# Autodesk Inventor assembly: Assembly6
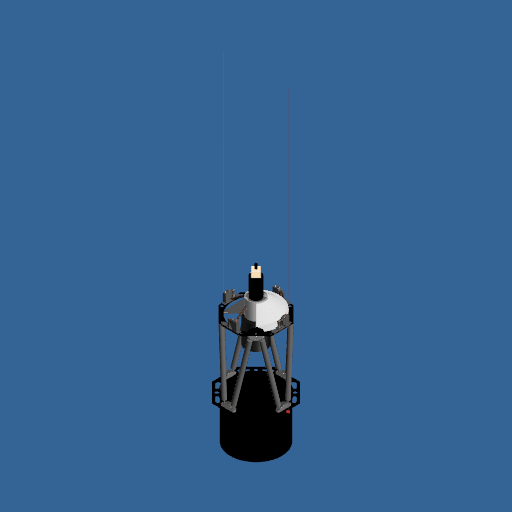
[picture p0: Inventor's stored thumbnail of the model, 512x512]
Saved by Autodesk Inventor 2026.2 (Build 302298000, 298)
## iProperties
Created: 2025-12-09
Part Number: Assembly6
Document SubType Name: Assembly
Designer: Thoma
Mass: 27295.5 g
Surface Area: 25498 cm^2
Volume: 10830.6 cm^3
Density: 2.52023 g/cm^3
Author: Thoma
## Documents named in this file (30)
- C:\Users\Thoma\OneDrive\Desktop\dir\telescope_cover\cover\derive_covers_v4.iam
- C:\Users\Thoma\OneDrive\Desktop\dir\telescope_cover\telescope\version_3\Telescope_End.ipt
- C:\Users\Thoma\OneDrive\Desktop\dir\telescope_cover\telescope\version_3\Triangle.ipt
- C:\Users\Thoma\OneDrive\Desktop\dir\telescope_cover\telescope\version_3\Triangle_Bracket_Top.ipt
- C:\Users\Thoma\OneDrive\Desktop\dir\telescope_cover\telescope\version_3\Carbon_Fibre.ipt
- C:\Users\Thoma\OneDrive\Desktop\dir\telescope_cover\telescope\version_3\5mm Screw.ipt
- C:\Users\Thoma\OneDrive\Desktop\dir\telescope_cover\telescope\version_3\35mm_bolt.ipt
- C:\Users\Thoma\OneDrive\Desktop\dir\telescope_cover\telescope\version_3\Triangle_Bracket_Bottom_MIR.ipt
- C:\Users\Thoma\OneDrive\Desktop\dir\telescope_cover\telescope\version_3\Telescope_Base.ipt
- C:\Users\Thoma\OneDrive\Desktop\dir\telescope_cover\telescope\version_3\Full_shaft_Simplify_3.ipt
- C:\Users\Thoma\OneDrive\Desktop\dir\telescope_cover\cover\Conic_Cover_Simplify_1.ipt
- C:\Users\Thoma\OneDrive\Desktop\dir\telescope_cover\telescope\version_3\30mm_bolt.ipt
- C:\Users\Thoma\OneDrive\Desktop\dir\telescope_cover\telescope\version_3\Baffle.ipt
- C:\Users\Thoma\OneDrive\Desktop\dir\telescope_cover\telescope\version_3\Bottom_End_Top.ipt
- C:\Users\Thoma\OneDrive\Desktop\dir\telescope_cover\cover\Cover_Upper_v3.ipt
- C:\Users\Thoma\OneDrive\Desktop\dir\telescope_cover\telescope\version_3\Laser.ipt
- C:\Users\Thoma\OneDrive\Desktop\dir\telescope_cover\cover\rod_v10.ipt
- C:\Users\Thoma\OneDrive\Desktop\dir\telescope_cover\servo\DSS-M15S Servo.ipt
- C:\Users\Thoma\OneDrive\Desktop\dir\telescope_cover\cover\Base_Plate_bottom.ipt
- C:\Users\Thoma\OneDrive\Desktop\dir\telescope_cover\cover\pawn.ipt
- C:\Users\Thoma\OneDrive\Desktop\dir\telescope_cover\cover\4mm_screw.ipt
- C:\Users\Thoma\OneDrive\Desktop\dir\telescope_cover\cover\6mm_washer_1mm.ipt
- C:\Users\Thoma\OneDrive\Desktop\dir\telescope_cover\cover\base_plate_v8.ipt
- C:\Users\Thoma\OneDrive\Desktop\dir\telescope_cover\screws\M2_Insert.ipt
- C:\Users\Thoma\OneDrive\Desktop\dir\telescope_cover\screws\Screw_DIN_912_M2x5F_A2.ipt
- C:\Users\Thoma\OneDrive\Desktop\dir\telescope_cover\screws\washer_bossard_m2-5_1170171.ipt
- C:\Users\Thoma\OneDrive\Desktop\dir\telescope_cover\screws\m4 threaded insert\m4 threaded insert\m4 threaded insert.ipt
- C:\Users\Thoma\OneDrive\Desktop\dir\telescope_cover\screws\M4 Washer - 9.0 x 0.9 - Black\M4 Washer - 9.0 x 0.9 - Black\M4 Washer - 9.0 x 0.9 - Black.ipt
- C:\Users\Thoma\OneDrive\Desktop\dir\telescope_cover\screws\Screw_DIN_912_M4x12F_A2\Screw_DIN_912_M4x12F_A2\Screw_DIN_912_M4x12F_A2.ipt
- C:\Users\Thoma\OneDrive\Desktop\dir\telescope_cover\cover\Cover_Lower_v3.ipt
## Components (140 placed, 29 different names)
1. M2_Insert:1 — Flush:222, Mate:437, Mate:444, Mate:446
2. Screw_DIN_912_M2x5F_A2:1 — Mate:444, Mate:447, Angle:138
3. washer_bossard_m2-5_1170171:1 — Mate:445, Mate:446, Mate:447
4. Screw_DIN_912_M2x5F_A2:2 — Mate:452, Angle:137
5. washer_bossard_m2-5_1170171:2 — Mate:449, Mate:450
6. M2_Insert:2 — Flush:452, Mate:451, Mate:452
7. pawn:5 — Mate:453, Mate:454, Angle:139
8. m4 threaded insert:1 — Mate:455, Flush:453
9. m4 threaded insert:2 — Mate:456, Flush:455
10. m4 threaded insert:3 — Mate:457, Flush:454, Mate:463
11. M4 Washer - 9.0 x 0.9 - Black:1 — Mate:458, Mate:463, Mate:464, Tangent:34
12. M4 Washer - 9.0 x 0.9 - Black:2 — Mate:459, Mate:462
13. M4 Washer - 9.0 x 0.9 - Black:3 — Mate:460, Mate:461, Mate:465
14. Cover_Upper_v3:1 — Mate:464, Mate:465, Mate:468, Mate:469, Mate:471, Tangent:34, Mate:472, Mate:473
15. Screw_DIN_912_M4x12F_A2:1 — Angle:140, Mate:470, Mate:471
16. Screw_DIN_912_M4x12F_A2:2 — Mate:468, Mate:469, Angle:141
17. Screw_DIN_912_M4x12F_A2:3 — Mate:472, Mate:473, Angle:142
18. M4 Washer - 9.0 x 0.9 - Black:4 — Mate:478, Mate:479, Tangent:35
19. M4 Washer - 9.0 x 0.9 - Black:5 — Mate:476, Mate:477
20. M4 Washer - 9.0 x 0.9 - Black:6 — Mate:474, Mate:475
21. Cover_Lower_v3:1 — Mate:480, Mate:481, Tangent:35, Mate:482, Mate:483, Mate:484, Mate:485, Mate:486, Mate:487
22. Screw_DIN_912_M4x12F_A2:4 — Mate:484, Mate:485, Angle:145
23. Screw_DIN_912_M4x12F_A2:5 — Mate:483, Mate:486, Angle:144
24. Screw_DIN_912_M4x12F_A2:6 — Mate:482, Mate:487, Angle:143
25. Laser:2 — Mate:214, Flush:220, Flush:221
26. Laser:1 — Mate:215, Flush:218, Flush:219
27. Baffle:1 — Mate:83
28. Carbon_Fibre:1 — Mate:7, Mate:11, Flush:1, Mate:12, Mate:13, Mate:14, Mate:15, Mate:62, Flush:2, Flush:3, Flush:4, Flush:5, Mate:83, Mate:92, Mate:93, Mate:96, Mate:97, Mate:98, Mate:100, Mate:123, Mate:124, Mate:125, Mate:213
29. Telescope_Base:1 — Mate:62, Angle:31, Mate:89, Mate:90, Angle:40, Mate:108, Mate:109, Angle:48, Mate:110, Mate:111, Angle:49, Mate:112, Mate:113, Angle:50, Mate:214, Mate:215, Flush:218, Flush:221
30. Telescope_End:1 — Mate:1, Mate:2, Angle:2, Mate:7, Mate:54, Mate:55, Angle:26, Angle:31, Mate:86, Mate:88, Mate:91, Angle:41, Mate:101, Angle:45, Angle:46, Mate:114, Mate:115, Angle:51, Mate:116, Mate:117, Angle:52, Mate:118, Mate:119, Angle:53, Mate:220, Mate:221, Mate:222, Mate:223, Mate:224, Mate:225, Mate:226, Mate:227, Mate:232, Mate:241, Mate:246, Mate:247, Mate:248, Mate:251, Mate:254, Mate:257
31. 30mm_bolt:9 — Mate:217, Mate:218, Angle:83
32. 30mm_bolt:10 — Mate:216, Mate:219, Angle:82
33. Triangle_Bracket_Top:5 — Mate:116, Mate:117, Angle:52, Mate:129, Flush:110, Angle:60
34. Triangle_Bracket_Top:4 — Mate:101, Angle:45, Angle:46, Mate:104, Mate:105, Mate:106, Flush:103, Angle:47
35. Triangle_Bracket_Top:3 — Mate:86, Mate:88, Mate:94, Angle:54, Angle:55, Mate:122, Flush:106, Angle:56
36. Triangle_Bracket_Top:1 — Mate:1, Mate:2, Angle:2, Mate:8, Mate:9, Angle:4, Mate:47, Angle:22, Mate:58
37. Triangle:1 — Mate:8, Mate:9, Angle:4, Mate:11, Flush:1, Angle:5, Angle:6, Mate:46, Mate:70, Mate:71
38. Triangle:5 — Mate:92, Mate:93, Mate:94, Mate:102, Mate:128, Flush:109, Angle:59, Mate:132, Flush:181, Angle:81
39. Triangle:6 — Mate:96, Mate:97, Mate:98, Flush:102, Angle:44, Mate:103, Mate:104, Mate:105, Mate:107
40. Triangle:7 — Mate:123, Mate:124, Mate:125, Mate:126, Flush:107, Angle:57, Mate:127, Flush:108, Angle:58, Mate:130, Mate:131
41. 35mm_bolt:6 — Mate:122, Flush:106, Angle:56
42. 35mm_bolt:7 — Mate:129, Flush:110, Angle:60
43. 35mm_bolt:4 — Mate:46, Mate:47, Angle:22
44. 35mm_bolt:5 — Mate:106, Flush:103, Angle:47
45. 5mm Screw:9 — Mate:100, Flush:102, Angle:44
46. 5mm Screw:13 — Mate:213, Flush:181, Angle:81
47. 5mm Screw:10 — Mate:126, Flush:107, Angle:57
48. 5mm Screw:2 — Mate:14, Mate:15, Angle:6
49. 5mm Screw:1 — Mate:12, Mate:13, Angle:5
50. 5mm Screw:11 — Mate:127, Flush:108, Angle:58
51. 5mm Screw:12 — Mate:128, Flush:109, Angle:59
52. Full_shaft_Simplify_3:1
53. Full_shaft_Simplify_3:2 — Tangent:26
54. Full_shaft_Simplify_3:3
55. Full_shaft_Simplify_3:4
56. Full_shaft_Simplify_3:5
57. Full_shaft_Simplify_3:6
58. Full_shaft_Simplify_3:7
59. Full_shaft_Simplify_3:8 — Tangent:31, Tangent:33
60. 30mm_bolt:7 — Mate:120, Flush:104, Angle:54
61. 30mm_bolt:1 — Mate:121, Flush:105, Angle:55
62. 30mm_bolt:8 — Mate:80, Flush:13, Angle:39
63. 30mm_bolt:6 — Mate:78, Flush:11, Angle:37
64. 30mm_bolt:3 — Mate:79, Flush:12, Angle:38
65. 30mm_bolt:2 — Mate:77, Flush:10, Angle:36
66. Triangle_Bracket_Bottom_MIR:4 — Mate:118, Mate:119, Angle:53, Mate:216, Mate:217, Mate:218, Mate:219, Angle:82, Angle:83
67. Triangle_Bracket_Bottom_MIR:3 — Mate:114, Mate:115, Angle:51, Mate:120, Flush:104, Mate:121, Flush:105
68. Triangle_Bracket_Bottom_MIR:2 — Mate:55, Mate:58, Angle:26, Mate:77, Flush:10, Angle:36, Mate:78, Flush:11, Angle:37, Tangent:31
69. Triangle_Bracket_Bottom_MIR:1 — Mate:54, Mate:79, Flush:12, Angle:38, Mate:80, Flush:13, Angle:39, Mate:91, Angle:41
70. Bottom_End_Top:4 — Mate:112, Mate:113, Angle:50, Tangent:26, Tangent:33
71. Bottom_End_Top:3 — Mate:110, Mate:111, Angle:49, Flush:219
72. Bottom_End_Top:2 — Mate:108, Mate:109, Angle:48
73. Bottom_End_Top:1 — Mate:89, Mate:90, Angle:40, Flush:220
74. Conic_Cover_Simplify_1:1 — Flush:2, Mate:131, Mate:132
75. Conic_Cover_Simplify_1:2 — Flush:3, Mate:102, Mate:103
76. Conic_Cover_Simplify_1:3 — Flush:4, Mate:70, Mate:107
77. Conic_Cover_Simplify_1:4 — Mate:71, Flush:5, Mate:130
78. pawn:1 — Mate:228, Mate:229, Angle:84, Mate:419
79. pawn:2 — Mate:235, Mate:238, Angle:86, Mate:403
80. pawn:4 — Mate:233, Mate:236, Angle:87, Mate:435
81. 4mm_screw:1 — Mate:230, Mate:231, Angle:85
82. 4mm_screw:2 — Mate:244, Mate:245, Angle:91
83. 4mm_screw:3 — Mate:242, Mate:243, Angle:90, Mate:385, Mate:454
84. 4mm_screw:4 — Mate:239, Mate:240, Angle:89
85. Base_Plate_bottom:1 — Mate:248, Mate:249, Mate:250, Mate:278, Mate:279, Angle:101, Mate:280, Mate:281, Angle:102, Mate:282, Mate:283, Angle:103
86. Base_Plate_bottom:2 — Mate:257, Mate:258, Mate:259, Mate:260, Mate:261, Mate:262, Mate:263, Angle:92, Mate:264, Angle:93, Mate:265, Angle:94
87. Base_Plate_bottom:3 — Mate:254, Mate:255, Mate:256, Mate:266, Mate:267, Angle:95, Mate:268, Mate:269, Angle:96, Mate:270, Mate:271, Angle:97
88. Base_Plate_bottom:4 — Mate:251, Mate:252, Mate:253, Mate:272, Mate:273, Angle:98, Mate:274, Mate:275, Angle:99, Mate:276, Mate:277, Angle:100
89. 4mm_screw:5 — Mate:262, Mate:263, Angle:92
90. 4mm_screw:6 — Mate:261, Mate:264, Angle:93
91. 4mm_screw:7 — Mate:260, Mate:265, Angle:94
92. 4mm_screw:8 — Mate:270, Mate:271, Angle:97
93. 4mm_screw:9 — Mate:268, Mate:269, Angle:96
94. 4mm_screw:10 — Mate:266, Mate:267, Angle:95
95. 4mm_screw:11 — Mate:276, Mate:277, Angle:100
96. 4mm_screw:12 — Mate:274, Mate:275, Angle:99
97. 4mm_screw:13 — Mate:272, Mate:273, Angle:98
98. 4mm_screw:14 — Mate:282, Mate:283, Angle:103
99. 4mm_screw:15 — Mate:280, Mate:281, Angle:102
100. 4mm_screw:16 — Mate:278, Mate:279, Angle:101
101. DSS-M15S Servo:1 — Mate:284, Mate:285, Mate:286, Mate:420
102. DSS-M15S Servo:2 — Mate:287, Mate:288, Mate:289, Mate:436
103. DSS-M15S Servo:3 — Mate:290, Mate:291, Mate:292, Mate:387, Mate:388
104. DSS-M15S Servo:4 — Mate:293, Mate:294, Mate:295, Mate:404, Flush:452
105. 6mm_washer_1mm:2 — Mate:297, Mate:303, Mate:311
106. 6mm_washer_1mm:3 — Mate:296, Mate:302, Mate:309
107. 4mm_screw:17 — Mate:310, Mate:311, Angle:107
108. 4mm_screw:18 — Mate:308, Mate:309, Angle:106
109. 6mm_washer_1mm:5 — Mate:315, Mate:317, Mate:324, Mate:325
110. 6mm_washer_1mm:6 — Mate:314, Mate:316, Mate:322, Mate:323
111. 6mm_washer_1mm:7 — Mate:313, Mate:319, Mate:326, Mate:327
112. 6mm_washer_1mm:8 — Mate:312, Mate:318, Mate:320, Mate:321
113. 4mm_screw:21 — Mate:326, Mate:327, Angle:111
114. 4mm_screw:22 — Mate:324, Mate:325, Angle:110
115. 4mm_screw:23 — Mate:322, Mate:323, Angle:109
116. 4mm_screw:24 — Mate:320, Mate:321, Angle:108
117. 6mm_washer_1mm:9 — Mate:341, Mate:343, Mate:349
118. 6mm_washer_1mm:10 — Mate:340, Mate:342, Mate:347
119. 6mm_washer_1mm:11 — Mate:339, Mate:345, Mate:353
120. 6mm_washer_1mm:12 — Mate:338, Mate:344, Mate:351
121. 4mm_screw:25 — Mate:350, Mate:351, Angle:114
122. 4mm_screw:26 — Mate:352, Mate:353, Angle:115
123. 4mm_screw:27 — Mate:348, Angle:113, Mate:349
124. 4mm_screw:28 — Mate:346, Mate:347, Angle:112
125. 6mm_washer_1mm:13 — Mate:360, Mate:361, Mate:364, Mate:365
126. 6mm_washer_1mm:14 — Mate:358, Mate:359, Mate:362, Mate:363
127. 6mm_washer_1mm:15 — Mate:356, Mate:357, Mate:368, Mate:369
128. 6mm_washer_1mm:16 — Mate:354, Mate:355, Mate:366, Mate:367
129. 4mm_screw:29 — Mate:368, Mate:369, Angle:119
130. 4mm_screw:30 — Mate:366, Mate:367, Angle:118
131. 4mm_screw:31 — Mate:364, Mate:365, Angle:117
132. 4mm_screw:32 — Mate:362, Mate:363, Angle:116
133. rod_v10:3 — Mate:387, Mate:388, Angle:136, Angle:139
134. rod_v10:2 — Mate:419, Mate:420, Angle:131, Mate:455, Flush:453, Mate:456, Mate:457, Flush:454, Flush:455, Mate:458, Mate:459, Mate:460, Mate:461, Mate:462, Angle:140, Mate:470, Angle:141, Angle:142
135. rod_v10:1 — Mate:403, Mate:404, Angle:127, Mate:474, Mate:475, Mate:476, Mate:477, Mate:478, Mate:479, Mate:480, Mate:481, Angle:143, Angle:144, Angle:145
136. rod_v10:4 — Mate:435, Angle:135, Mate:436
137. base_plate_v8:1 — Mate:223, Mate:227, Mate:235, Mate:238, Angle:86, Mate:244, Mate:245, Angle:91, Mate:246, Mate:249, Mate:250, Mate:293, Mate:294, Mate:295, Mate:296, Mate:297, Mate:302, Mate:303, Mate:308, Angle:106, Mate:310, Angle:107, Angle:127, Flush:222, Mate:437, Mate:445, Mate:449, Mate:450, Mate:451, Angle:137, Angle:138
138. base_plate_v8:2 — Mate:220, Mate:225, Mate:233, Mate:236, Angle:87, Mate:239, Mate:240, Angle:89, Mate:241, Mate:255, Mate:256, Mate:287, Mate:288, Mate:289, Mate:338, Mate:339, Mate:340, Mate:341, Mate:342, Mate:343, Mate:344, Mate:345, Mate:346, Angle:112, Mate:348, Angle:113, Mate:350, Angle:114, Mate:352, Angle:115, Angle:135
139. base_plate_v8:3 — Mate:221, Mate:226, Mate:242, Mate:243, Angle:90, Mate:247, Mate:252, Mate:253, Mate:290, Mate:291, Mate:292, Mate:354, Mate:355, Mate:356, Mate:357, Mate:358, Mate:359, Mate:360, Mate:361, Angle:116, Angle:117, Angle:118, Angle:119, Mate:385, Angle:136, Mate:453
140. base_plate_v8:4 — Mate:222, Mate:224, Mate:228, Mate:229, Angle:84, Mate:230, Mate:231, Angle:85, Mate:232, Mate:258, Mate:259, Mate:284, Mate:285, Mate:286, Mate:312, Mate:313, Mate:314, Mate:315, Mate:316, Mate:317, Mate:318, Mate:319, Angle:108, Angle:109, Angle:110, Angle:111, Angle:131
## Relationships (368: Mate 256, Angle 79, Flush 28, Tangent 5)
- Mate:1: Telescope_End:1 ↔ Triangle_Bracket_Top:1
- Mate:2: Telescope_End:1 ↔ Triangle_Bracket_Top:1
- Angle:2 (0 deg): Telescope_End:1 ↔ Triangle_Bracket_Top:1
- Mate:7: Carbon_Fibre:1 ↔ Telescope_End:1
- Mate:8: Triangle_Bracket_Top:1 ↔ Triangle:1
- Mate:9: Triangle_Bracket_Top:1 ↔ Triangle:1
- Angle:4 (0 deg): Triangle_Bracket_Top:1 ↔ Triangle:1
- Mate:11: Carbon_Fibre:1 ↔ Triangle:1
- Flush:1: Carbon_Fibre:1 ↔ Triangle:1
- Mate:12: Carbon_Fibre:1 ↔ 5mm Screw:1
- Mate:13: Carbon_Fibre:1 ↔ 5mm Screw:1
- Angle:5 (0 deg): Triangle:1 ↔ 5mm Screw:1
- Mate:14: Carbon_Fibre:1 ↔ 5mm Screw:2
- Mate:15: Carbon_Fibre:1 ↔ 5mm Screw:2
- Angle:6 (0 deg): Triangle:1 ↔ 5mm Screw:2
- Mate:46: Triangle:1 ↔ 35mm_bolt:4
- Mate:47: Triangle_Bracket_Top:1 ↔ 35mm_bolt:4
- Angle:22 (0 deg): Triangle_Bracket_Top:1 ↔ 35mm_bolt:4
- Mate:54: Telescope_End:1 ↔ Triangle_Bracket_Bottom_MIR:1
- Mate:55: Telescope_End:1 ↔ Triangle_Bracket_Bottom_MIR:2
- Mate:58: Triangle_Bracket_Top:1 ↔ Triangle_Bracket_Bottom_MIR:2
- Angle:26 (0 deg): Telescope_End:1 ↔ Triangle_Bracket_Bottom_MIR:2
- Mate:62: Carbon_Fibre:1 ↔ Telescope_Base:1
- Angle:31 (0 deg): Telescope_Base:1 ↔ Telescope_End:1
- Flush:2: Carbon_Fibre:1 ↔ Conic_Cover_Simplify_1:1
- Flush:3: Carbon_Fibre:1 ↔ Conic_Cover_Simplify_1:2
- Flush:4: Carbon_Fibre:1 ↔ Conic_Cover_Simplify_1:3
- Mate:70: Triangle:1 ↔ Conic_Cover_Simplify_1:3
- Mate:71: Triangle:1 ↔ Conic_Cover_Simplify_1:4
- Flush:5: Carbon_Fibre:1 ↔ Conic_Cover_Simplify_1:4
- Mate:77: 30mm_bolt:2 ↔ Triangle_Bracket_Bottom_MIR:2
- Flush:10: 30mm_bolt:2 ↔ Triangle_Bracket_Bottom_MIR:2
- Angle:36 (0 deg): 30mm_bolt:2 ↔ Triangle_Bracket_Bottom_MIR:2
- Mate:78: 30mm_bolt:6 ↔ Triangle_Bracket_Bottom_MIR:2
- Flush:11: 30mm_bolt:6 ↔ Triangle_Bracket_Bottom_MIR:2
- Angle:37 (0 deg): 30mm_bolt:6 ↔ Triangle_Bracket_Bottom_MIR:2
- Mate:79: 30mm_bolt:3 ↔ Triangle_Bracket_Bottom_MIR:1
- Flush:12: 30mm_bolt:3 ↔ Triangle_Bracket_Bottom_MIR:1
- Angle:38 (0 deg): 30mm_bolt:3 ↔ Triangle_Bracket_Bottom_MIR:1
- Mate:80: 30mm_bolt:8 ↔ Triangle_Bracket_Bottom_MIR:1
- Flush:13: 30mm_bolt:8 ↔ Triangle_Bracket_Bottom_MIR:1
- Angle:39 (0 deg): 30mm_bolt:8 ↔ Triangle_Bracket_Bottom_MIR:1
- Mate:83: Baffle:1 ↔ Carbon_Fibre:1
- Mate:86: Telescope_End:1 ↔ Triangle_Bracket_Top:3
- Mate:88: Telescope_End:1 ↔ Triangle_Bracket_Top:3
- Mate:89: Telescope_Base:1 ↔ Bottom_End_Top:1
- Mate:90: Telescope_Base:1 ↔ Bottom_End_Top:1
- Angle:40 (0 deg): Telescope_Base:1 ↔ Bottom_End_Top:1
- Mate:91: Telescope_End:1 ↔ Triangle_Bracket_Bottom_MIR:1
- Angle:41 (0 deg): Telescope_End:1 ↔ Triangle_Bracket_Bottom_MIR:1
- Mate:92: Carbon_Fibre:1 ↔ Triangle:5
- Mate:93: Carbon_Fibre:1 ↔ Triangle:5
- Mate:94: Triangle_Bracket_Top:3 ↔ Triangle:5
- Mate:96: Carbon_Fibre:1 ↔ Triangle:6
- Mate:97: Carbon_Fibre:1 ↔ Triangle:6
- Mate:98: Carbon_Fibre:1 ↔ Triangle:6
- Mate:100: Carbon_Fibre:1 ↔ 5mm Screw:9
- Flush:102: Triangle:6 ↔ 5mm Screw:9
- Angle:44 (0 deg): Triangle:6 ↔ 5mm Screw:9
- Mate:101: Telescope_End:1 ↔ Triangle_Bracket_Top:4
- Angle:45 (0 deg): Telescope_End:1 ↔ Triangle_Bracket_Top:4
- Mate:102: Triangle:5 ↔ Conic_Cover_Simplify_1:2
- Mate:103: Triangle:6 ↔ Conic_Cover_Simplify_1:2
- Angle:46 (0 deg): Telescope_End:1 ↔ Triangle_Bracket_Top:4
- Mate:104: Triangle_Bracket_Top:4 ↔ Triangle:6
- Mate:105: Triangle_Bracket_Top:4 ↔ Triangle:6
- Mate:106: Triangle_Bracket_Top:4 ↔ 35mm_bolt:5
- Flush:103: Triangle_Bracket_Top:4 ↔ 35mm_bolt:5
- Angle:47 (0 deg): Triangle_Bracket_Top:4 ↔ 35mm_bolt:5
- Mate:107: Triangle:6 ↔ Conic_Cover_Simplify_1:3
- Mate:108: Telescope_Base:1 ↔ Bottom_End_Top:2
- Mate:109: Telescope_Base:1 ↔ Bottom_End_Top:2
- Angle:48 (0 deg): Telescope_Base:1 ↔ Bottom_End_Top:2
- Mate:110: Telescope_Base:1 ↔ Bottom_End_Top:3
- Mate:111: Telescope_Base:1 ↔ Bottom_End_Top:3
- Angle:49 (0 deg): Telescope_Base:1 ↔ Bottom_End_Top:3
- Mate:112: Telescope_Base:1 ↔ Bottom_End_Top:4
- Mate:113: Telescope_Base:1 ↔ Bottom_End_Top:4
- Angle:50 (0 deg): Telescope_Base:1 ↔ Bottom_End_Top:4
- Mate:114: Telescope_End:1 ↔ Triangle_Bracket_Bottom_MIR:3
- Mate:115: Telescope_End:1 ↔ Triangle_Bracket_Bottom_MIR:3
- Angle:51 (0 deg): Telescope_End:1 ↔ Triangle_Bracket_Bottom_MIR:3
- Mate:116: Telescope_End:1 ↔ Triangle_Bracket_Top:5
- Mate:117: Telescope_End:1 ↔ Triangle_Bracket_Top:5
- Angle:52 (0 deg): Telescope_End:1 ↔ Triangle_Bracket_Top:5
- Mate:118: Telescope_End:1 ↔ Triangle_Bracket_Bottom_MIR:4
- Mate:119: Telescope_End:1 ↔ Triangle_Bracket_Bottom_MIR:4
- Angle:53 (0 deg): Telescope_End:1 ↔ Triangle_Bracket_Bottom_MIR:4
- Mate:120: 30mm_bolt:7 ↔ Triangle_Bracket_Bottom_MIR:3
- Flush:104: 30mm_bolt:7 ↔ Triangle_Bracket_Bottom_MIR:3
- Angle:54 (0 deg): Triangle_Bracket_Top:3 ↔ 30mm_bolt:7
- Mate:121: 30mm_bolt:1 ↔ Triangle_Bracket_Bottom_MIR:3
- Flush:105: 30mm_bolt:1 ↔ Triangle_Bracket_Bottom_MIR:3
- Angle:55 (0 deg): Triangle_Bracket_Top:3 ↔ 30mm_bolt:1
- Mate:122: Triangle_Bracket_Top:3 ↔ 35mm_bolt:6
- Flush:106: Triangle_Bracket_Top:3 ↔ 35mm_bolt:6
- Angle:56 (0 deg): Triangle_Bracket_Top:3 ↔ 35mm_bolt:6
- Mate:123: Carbon_Fibre:1 ↔ Triangle:7
- Mate:124: Carbon_Fibre:1 ↔ Triangle:7
- Mate:125: Carbon_Fibre:1 ↔ Triangle:7
- Mate:126: Triangle:7 ↔ 5mm Screw:10
- Flush:107: Triangle:7 ↔ 5mm Screw:10
- Angle:57 (0 deg): Triangle:7 ↔ 5mm Screw:10
- Mate:127: Triangle:7 ↔ 5mm Screw:11
- Flush:108: Triangle:7 ↔ 5mm Screw:11
- Angle:58 (0 deg): Triangle:7 ↔ 5mm Screw:11
- Mate:128: Triangle:5 ↔ 5mm Screw:12
- Flush:109: Triangle:5 ↔ 5mm Screw:12
- Angle:59 (0 deg): Triangle:5 ↔ 5mm Screw:12
- Mate:129: Triangle_Bracket_Top:5 ↔ 35mm_bolt:7
- Flush:110: Triangle_Bracket_Top:5 ↔ 35mm_bolt:7
- Angle:60 (0 deg): Triangle_Bracket_Top:5 ↔ 35mm_bolt:7
- Mate:130: Triangle:7 ↔ Conic_Cover_Simplify_1:4
- Mate:131: Triangle:7 ↔ Conic_Cover_Simplify_1:1
- Mate:132: Triangle:5 ↔ Conic_Cover_Simplify_1:1
- Mate:213: Carbon_Fibre:1 ↔ 5mm Screw:13
- Flush:181: Triangle:5 ↔ 5mm Screw:13
- Angle:81 (0 deg): Triangle:5 ↔ 5mm Screw:13
- Mate:214: Laser:2 ↔ Telescope_Base:1
- Mate:215: Laser:1 ↔ Telescope_Base:1
- Flush:218: Laser:1 ↔ Telescope_Base:1
- Flush:219 (39.316 mm): Laser:1 ↔ Bottom_End_Top:3
- Flush:220 (39.316 mm): Laser:2 ↔ Bottom_End_Top:1
- Flush:221: Laser:2 ↔ Telescope_Base:1
- Tangent:26: Full_shaft_Simplify_3:2 ↔ Bottom_End_Top:4
- Tangent:31: Full_shaft_Simplify_3:8 ↔ Triangle_Bracket_Bottom_MIR:2
- Tangent:33: Full_shaft_Simplify_3:8 ↔ Bottom_End_Top:4
- Mate:216: 30mm_bolt:10 ↔ Triangle_Bracket_Bottom_MIR:4
- Mate:217: 30mm_bolt:9 ↔ Triangle_Bracket_Bottom_MIR:4
- Mate:218: 30mm_bolt:9 ↔ Triangle_Bracket_Bottom_MIR:4
- Mate:219: 30mm_bolt:10 ↔ Triangle_Bracket_Bottom_MIR:4
- Angle:82 (0 deg): 30mm_bolt:10 ↔ Triangle_Bracket_Bottom_MIR:4
- Angle:83 (0 deg): 30mm_bolt:9 ↔ Triangle_Bracket_Bottom_MIR:4
- Mate:220: Telescope_End:1 ↔ base_plate_v8:2
- Mate:221: Telescope_End:1 ↔ base_plate_v8:3
- Mate:222: Telescope_End:1 ↔ base_plate_v8:4
- Mate:223: Telescope_End:1 ↔ base_plate_v8:1
- Mate:224: Telescope_End:1 ↔ base_plate_v8:4
- Mate:225: Telescope_End:1 ↔ base_plate_v8:2
- Mate:226: Telescope_End:1 ↔ base_plate_v8:3
- Mate:227: Telescope_End:1 ↔ base_plate_v8:1
- Mate:228: pawn:1 ↔ base_plate_v8:4
- Mate:229: pawn:1 ↔ base_plate_v8:4
- Angle:84 (180 deg): pawn:1 ↔ base_plate_v8:4
- Mate:230: 4mm_screw:1 ↔ base_plate_v8:4
- Mate:231: 4mm_screw:1 ↔ base_plate_v8:4
- Angle:85 (0 deg): 4mm_screw:1 ↔ base_plate_v8:4
- Mate:232: Telescope_End:1 ↔ base_plate_v8:4
- Mate:233: pawn:4 ↔ base_plate_v8:2
- Mate:235: pawn:2 ↔ base_plate_v8:1
- Mate:236: pawn:4 ↔ base_plate_v8:2
- Mate:238: pawn:2 ↔ base_plate_v8:1
- Angle:86 (0 deg): pawn:2 ↔ base_plate_v8:1
- Angle:87 (0 deg): pawn:4 ↔ base_plate_v8:2
- Mate:239: 4mm_screw:4 ↔ base_plate_v8:2
- Mate:240: 4mm_screw:4 ↔ base_plate_v8:2
- Angle:89 (0 deg): 4mm_screw:4 ↔ base_plate_v8:2
- Mate:241: Telescope_End:1 ↔ base_plate_v8:2
- Mate:242: 4mm_screw:3 ↔ base_plate_v8:3
- Mate:243: 4mm_screw:3 ↔ base_plate_v8:3
- Angle:90 (0 deg): 4mm_screw:3 ↔ base_plate_v8:3
- Mate:244: 4mm_screw:2 ↔ base_plate_v8:1
- Mate:245: 4mm_screw:2 ↔ base_plate_v8:1
- Angle:91 (0 deg): 4mm_screw:2 ↔ base_plate_v8:1
- Mate:246: Telescope_End:1 ↔ base_plate_v8:1
- Mate:247: Telescope_End:1 ↔ base_plate_v8:3
- Mate:248: Telescope_End:1 ↔ Base_Plate_bottom:1
- Mate:249: Base_Plate_bottom:1 ↔ base_plate_v8:1
- Mate:250: Base_Plate_bottom:1 ↔ base_plate_v8:1
- Mate:251: Telescope_End:1 ↔ Base_Plate_bottom:4
- Mate:252: Base_Plate_bottom:4 ↔ base_plate_v8:3
- Mate:253: Base_Plate_bottom:4 ↔ base_plate_v8:3
- Mate:254: Telescope_End:1 ↔ Base_Plate_bottom:3
- Mate:255: Base_Plate_bottom:3 ↔ base_plate_v8:2
- Mate:256: Base_Plate_bottom:3 ↔ base_plate_v8:2
- Mate:257: Telescope_End:1 ↔ Base_Plate_bottom:2
- Mate:258: Base_Plate_bottom:2 ↔ base_plate_v8:4
- Mate:259: Base_Plate_bottom:2 ↔ base_plate_v8:4
- Mate:260: Base_Plate_bottom:2 ↔ 4mm_screw:7
- Mate:261: Base_Plate_bottom:2 ↔ 4mm_screw:6
- Mate:262: Base_Plate_bottom:2 ↔ 4mm_screw:5
- Mate:263: Base_Plate_bottom:2 ↔ 4mm_screw:5
- Angle:92 (0 deg): Base_Plate_bottom:2 ↔ 4mm_screw:5
- Mate:264: Base_Plate_bottom:2 ↔ 4mm_screw:6
- Angle:93 (0 deg): Base_Plate_bottom:2 ↔ 4mm_screw:6
- Mate:265: Base_Plate_bottom:2 ↔ 4mm_screw:7
- Angle:94 (0 deg): Base_Plate_bottom:2 ↔ 4mm_screw:7
- Mate:266: Base_Plate_bottom:3 ↔ 4mm_screw:10
- Mate:267: Base_Plate_bottom:3 ↔ 4mm_screw:10
- Angle:95 (0 deg): Base_Plate_bottom:3 ↔ 4mm_screw:10
- Mate:268: Base_Plate_bottom:3 ↔ 4mm_screw:9
- Mate:269: Base_Plate_bottom:3 ↔ 4mm_screw:9
- Angle:96 (0 deg): Base_Plate_bottom:3 ↔ 4mm_screw:9
- Mate:270: Base_Plate_bottom:3 ↔ 4mm_screw:8
- Mate:271: Base_Plate_bottom:3 ↔ 4mm_screw:8
- Angle:97 (0 deg): Base_Plate_bottom:3 ↔ 4mm_screw:8
- Mate:272: Base_Plate_bottom:4 ↔ 4mm_screw:13
- Mate:273: Base_Plate_bottom:4 ↔ 4mm_screw:13
- Angle:98 (0 deg): Base_Plate_bottom:4 ↔ 4mm_screw:13
- Mate:274: Base_Plate_bottom:4 ↔ 4mm_screw:12
- Mate:275: Base_Plate_bottom:4 ↔ 4mm_screw:12
- Angle:99 (0 deg): Base_Plate_bottom:4 ↔ 4mm_screw:12
- Mate:276: Base_Plate_bottom:4 ↔ 4mm_screw:11
- Mate:277: Base_Plate_bottom:4 ↔ 4mm_screw:11
- Angle:100 (0 deg): Base_Plate_bottom:4 ↔ 4mm_screw:11
- Mate:278: Base_Plate_bottom:1 ↔ 4mm_screw:16
- Mate:279: Base_Plate_bottom:1 ↔ 4mm_screw:16
- Angle:101 (0 deg): Base_Plate_bottom:1 ↔ 4mm_screw:16
- Mate:280: Base_Plate_bottom:1 ↔ 4mm_screw:15
- Mate:281: Base_Plate_bottom:1 ↔ 4mm_screw:15
- Angle:102 (0 deg): Base_Plate_bottom:1 ↔ 4mm_screw:15
- Mate:282: Base_Plate_bottom:1 ↔ 4mm_screw:14
- Mate:283: Base_Plate_bottom:1 ↔ 4mm_screw:14
- Angle:103 (0 deg): Base_Plate_bottom:1 ↔ 4mm_screw:14
- Mate:284 (1.1 mm): DSS-M15S Servo:1 ↔ base_plate_v8:4
- Mate:285: DSS-M15S Servo:1 ↔ base_plate_v8:4
- Mate:286: DSS-M15S Servo:1 ↔ base_plate_v8:4
- Mate:287 (1.1 mm): DSS-M15S Servo:2 ↔ base_plate_v8:2
- Mate:288: DSS-M15S Servo:2 ↔ base_plate_v8:2
- Mate:289: DSS-M15S Servo:2 ↔ base_plate_v8:2
- Mate:290 (1.1 mm): DSS-M15S Servo:3 ↔ base_plate_v8:3
- Mate:291: DSS-M15S Servo:3 ↔ base_plate_v8:3
- Mate:292: DSS-M15S Servo:3 ↔ base_plate_v8:3
- Mate:293 (1.1 mm): DSS-M15S Servo:4 ↔ base_plate_v8:1
- Mate:294: DSS-M15S Servo:4 ↔ base_plate_v8:1
- Mate:295: DSS-M15S Servo:4 ↔ base_plate_v8:1
- Mate:296: 6mm_washer_1mm:3 ↔ base_plate_v8:1
- Mate:297: 6mm_washer_1mm:2 ↔ base_plate_v8:1
- Mate:302: 6mm_washer_1mm:3 ↔ base_plate_v8:1
- Mate:303: 6mm_washer_1mm:2 ↔ base_plate_v8:1
- Mate:308: 4mm_screw:18 ↔ base_plate_v8:1
- Mate:309: 6mm_washer_1mm:3 ↔ 4mm_screw:18
- Angle:106 (0 deg): 4mm_screw:18 ↔ base_plate_v8:1
- Mate:310: 4mm_screw:17 ↔ base_plate_v8:1
- Mate:311: 6mm_washer_1mm:2 ↔ 4mm_screw:17
- Angle:107 (0 deg): 4mm_screw:17 ↔ base_plate_v8:1
- Mate:312: 6mm_washer_1mm:8 ↔ base_plate_v8:4
- Mate:313: 6mm_washer_1mm:7 ↔ base_plate_v8:4
- Mate:314: 6mm_washer_1mm:6 ↔ base_plate_v8:4
- Mate:315: 6mm_washer_1mm:5 ↔ base_plate_v8:4
- Mate:316: 6mm_washer_1mm:6 ↔ base_plate_v8:4
- Mate:317: 6mm_washer_1mm:5 ↔ base_plate_v8:4
- Mate:318: 6mm_washer_1mm:8 ↔ base_plate_v8:4
- Mate:319: 6mm_washer_1mm:7 ↔ base_plate_v8:4
- Mate:320: 6mm_washer_1mm:8 ↔ 4mm_screw:24
- Mate:321: 6mm_washer_1mm:8 ↔ 4mm_screw:24
- Angle:108 (0 deg): 4mm_screw:24 ↔ base_plate_v8:4
- Mate:322: 6mm_washer_1mm:6 ↔ 4mm_screw:23
- Mate:323: 6mm_washer_1mm:6 ↔ 4mm_screw:23
- Angle:109 (0 deg): 4mm_screw:23 ↔ base_plate_v8:4
- Mate:324: 6mm_washer_1mm:5 ↔ 4mm_screw:22
- Mate:325: 6mm_washer_1mm:5 ↔ 4mm_screw:22
- Angle:110 (0 deg): 4mm_screw:22 ↔ base_plate_v8:4
- Mate:326: 6mm_washer_1mm:7 ↔ 4mm_screw:21
- Mate:327: 6mm_washer_1mm:7 ↔ 4mm_screw:21
- Angle:111 (0 deg): 4mm_screw:21 ↔ base_plate_v8:4
- Mate:338: 6mm_washer_1mm:12 ↔ base_plate_v8:2
- Mate:339: 6mm_washer_1mm:11 ↔ base_plate_v8:2
- Mate:340: 6mm_washer_1mm:10 ↔ base_plate_v8:2
- Mate:341: 6mm_washer_1mm:9 ↔ base_plate_v8:2
- Mate:342: 6mm_washer_1mm:10 ↔ base_plate_v8:2
- Mate:343: 6mm_washer_1mm:9 ↔ base_plate_v8:2
- Mate:344: 6mm_washer_1mm:12 ↔ base_plate_v8:2
- Mate:345: 6mm_washer_1mm:11 ↔ base_plate_v8:2
- Mate:346: 4mm_screw:28 ↔ base_plate_v8:2
- Mate:347: 6mm_washer_1mm:10 ↔ 4mm_screw:28
- Angle:112 (0 deg): 4mm_screw:28 ↔ base_plate_v8:2
- Mate:348: 4mm_screw:27 ↔ base_plate_v8:2
- Angle:113 (0 deg): 4mm_screw:27 ↔ base_plate_v8:2
- Mate:349: 6mm_washer_1mm:9 ↔ 4mm_screw:27
- Mate:350: 4mm_screw:25 ↔ base_plate_v8:2
- Mate:351: 6mm_washer_1mm:12 ↔ 4mm_screw:25
- Angle:114 (0 deg): 4mm_screw:25 ↔ base_plate_v8:2
- Mate:352: 4mm_screw:26 ↔ base_plate_v8:2
- Mate:353: 6mm_washer_1mm:11 ↔ 4mm_screw:26
- Angle:115 (0 deg): 4mm_screw:26 ↔ base_plate_v8:2
- Mate:354: 6mm_washer_1mm:16 ↔ base_plate_v8:3
- Mate:355: 6mm_washer_1mm:16 ↔ base_plate_v8:3
- Mate:356: 6mm_washer_1mm:15 ↔ base_plate_v8:3
- Mate:357: 6mm_washer_1mm:15 ↔ base_plate_v8:3
- Mate:358: 6mm_washer_1mm:14 ↔ base_plate_v8:3
- Mate:359: 6mm_washer_1mm:14 ↔ base_plate_v8:3
- Mate:360: 6mm_washer_1mm:13 ↔ base_plate_v8:3
- Mate:361: 6mm_washer_1mm:13 ↔ base_plate_v8:3
- Mate:362: 6mm_washer_1mm:14 ↔ 4mm_screw:32
- Mate:363: 6mm_washer_1mm:14 ↔ 4mm_screw:32
- Angle:116 (0 deg): 4mm_screw:32 ↔ base_plate_v8:3
- Mate:364: 6mm_washer_1mm:13 ↔ 4mm_screw:31
- Mate:365: 6mm_washer_1mm:13 ↔ 4mm_screw:31
- Angle:117 (0 deg): 4mm_screw:31 ↔ base_plate_v8:3
- Mate:366: 6mm_washer_1mm:16 ↔ 4mm_screw:30
- Mate:367: 6mm_washer_1mm:16 ↔ 4mm_screw:30
- Angle:118 (0 deg): 4mm_screw:30 ↔ base_plate_v8:3
- Mate:368: 6mm_washer_1mm:15 ↔ 4mm_screw:29
- Mate:369: 6mm_washer_1mm:15 ↔ 4mm_screw:29
- Angle:119 (0 deg): 4mm_screw:29 ↔ base_plate_v8:3
- Mate:385: 4mm_screw:3 ↔ base_plate_v8:3
- Mate:387: DSS-M15S Servo:3 ↔ rod_v10:3
- Mate:388: DSS-M15S Servo:3 ↔ rod_v10:3
- Mate:403: pawn:2 ↔ rod_v10:1
- Mate:404: DSS-M15S Servo:4 ↔ rod_v10:1
- Angle:127 (232.647 deg): rod_v10:1 ↔ base_plate_v8:1
- Mate:419: pawn:1 ↔ rod_v10:2
- Mate:420: DSS-M15S Servo:1 ↔ rod_v10:2
- Angle:131 (127.357 deg): rod_v10:2 ↔ base_plate_v8:4
- Mate:435: pawn:4 ↔ rod_v10:4
- Angle:135 (127.357 deg): rod_v10:4 ↔ base_plate_v8:2
- Mate:436: DSS-M15S Servo:2 ↔ rod_v10:4
- Angle:136 (127.357 deg): rod_v10:3 ↔ base_plate_v8:3
- Flush:222 (0.05 mm): M2_Insert:1 ↔ base_plate_v8:1
- Mate:437: M2_Insert:1 ↔ base_plate_v8:1
- Mate:444: M2_Insert:1 ↔ Screw_DIN_912_M2x5F_A2:1
- Mate:445: washer_bossard_m2-5_1170171:1 ↔ base_plate_v8:1
- Mate:446: M2_Insert:1 ↔ washer_bossard_m2-5_1170171:1
- Mate:447: Screw_DIN_912_M2x5F_A2:1 ↔ washer_bossard_m2-5_1170171:1
- [Mate]: Screw_DIN_912_M2x5F_A2:2 ↔ washer_bossard_m2-5_1170171:2
- Mate:449: washer_bossard_m2-5_1170171:2 ↔ base_plate_v8:1
- Mate:450: washer_bossard_m2-5_1170171:2 ↔ base_plate_v8:1
- Flush:452 (0.05 mm): M2_Insert:2 ↔ DSS-M15S Servo:4
- Mate:451: M2_Insert:2 ↔ base_plate_v8:1
- Mate:452: Screw_DIN_912_M2x5F_A2:2 ↔ M2_Insert:2
- Angle:137 (0 deg): Screw_DIN_912_M2x5F_A2:2 ↔ base_plate_v8:1
- Angle:138 (0 deg): Screw_DIN_912_M2x5F_A2:1 ↔ base_plate_v8:1
- Mate:453: pawn:5 ↔ base_plate_v8:3
- Mate:454: pawn:5 ↔ 4mm_screw:3
- Angle:139 (180 deg): pawn:5 ↔ rod_v10:3
- Mate:455: m4 threaded insert:1 ↔ rod_v10:2
- Flush:453 (0.2 mm): m4 threaded insert:1 ↔ rod_v10:2
- Mate:456: m4 threaded insert:2 ↔ rod_v10:2
- Mate:457: m4 threaded insert:3 ↔ rod_v10:2
- Flush:454 (0.2 mm): m4 threaded insert:3 ↔ rod_v10:2
- Flush:455 (0.2 mm): m4 threaded insert:2 ↔ rod_v10:2
- Mate:458: M4 Washer - 9.0 x 0.9 - Black:1 ↔ rod_v10:2
- Mate:459: M4 Washer - 9.0 x 0.9 - Black:2 ↔ rod_v10:2
- Mate:460: M4 Washer - 9.0 x 0.9 - Black:3 ↔ rod_v10:2
- Mate:461: M4 Washer - 9.0 x 0.9 - Black:3 ↔ rod_v10:2
- Mate:462: M4 Washer - 9.0 x 0.9 - Black:2 ↔ rod_v10:2
- Mate:463: m4 threaded insert:3 ↔ M4 Washer - 9.0 x 0.9 - Black:1
- Mate:464: M4 Washer - 9.0 x 0.9 - Black:1 ↔ Cover_Upper_v3:1
- Mate:465: M4 Washer - 9.0 x 0.9 - Black:3 ↔ Cover_Upper_v3:1
- Angle:140 (0 deg): Screw_DIN_912_M4x12F_A2:1 ↔ rod_v10:2
- Mate:468: Cover_Upper_v3:1 ↔ Screw_DIN_912_M4x12F_A2:2
- Mate:469: Cover_Upper_v3:1 ↔ Screw_DIN_912_M4x12F_A2:2
- Mate:470: Screw_DIN_912_M4x12F_A2:1 ↔ rod_v10:2
- Mate:471: Cover_Upper_v3:1 ↔ Screw_DIN_912_M4x12F_A2:1
- Tangent:34: M4 Washer - 9.0 x 0.9 - Black:1 ↔ Cover_Upper_v3:1
- Angle:141 (0 deg): Screw_DIN_912_M4x12F_A2:2 ↔ rod_v10:2
- Mate:472: Cover_Upper_v3:1 ↔ Screw_DIN_912_M4x12F_A2:3
- Mate:473: Cover_Upper_v3:1 ↔ Screw_DIN_912_M4x12F_A2:3
- Angle:142 (0 deg): Screw_DIN_912_M4x12F_A2:3 ↔ rod_v10:2
- Mate:474: M4 Washer - 9.0 x 0.9 - Black:6 ↔ rod_v10:1
- Mate:475: M4 Washer - 9.0 x 0.9 - Black:6 ↔ rod_v10:1
- Mate:476: M4 Washer - 9.0 x 0.9 - Black:5 ↔ rod_v10:1
- Mate:477: M4 Washer - 9.0 x 0.9 - Black:5 ↔ rod_v10:1
- Mate:478: M4 Washer - 9.0 x 0.9 - Black:4 ↔ rod_v10:1
- Mate:479: M4 Washer - 9.0 x 0.9 - Black:4 ↔ rod_v10:1
- Mate:480: Cover_Lower_v3:1 ↔ rod_v10:1
- Mate:481: Cover_Lower_v3:1 ↔ rod_v10:1
- Tangent:35: M4 Washer - 9.0 x 0.9 - Black:4 ↔ Cover_Lower_v3:1
- Mate:482: Cover_Lower_v3:1 ↔ Screw_DIN_912_M4x12F_A2:6
- Mate:483: Cover_Lower_v3:1 ↔ Screw_DIN_912_M4x12F_A2:5
- Mate:484: Cover_Lower_v3:1 ↔ Screw_DIN_912_M4x12F_A2:4
- Mate:485: Cover_Lower_v3:1 ↔ Screw_DIN_912_M4x12F_A2:4
- Mate:486: Cover_Lower_v3:1 ↔ Screw_DIN_912_M4x12F_A2:5
- Mate:487: Cover_Lower_v3:1 ↔ Screw_DIN_912_M4x12F_A2:6
- Angle:143 (0 deg): Screw_DIN_912_M4x12F_A2:6 ↔ rod_v10:1
- Angle:144 (0 deg): Screw_DIN_912_M4x12F_A2:5 ↔ rod_v10:1
- Angle:145 (0 deg): Screw_DIN_912_M4x12F_A2:4 ↔ rod_v10:1
## Named parameters: d1329_d1328 = 0 mm
